# Autodesk Inventor assembly: CircuitCell
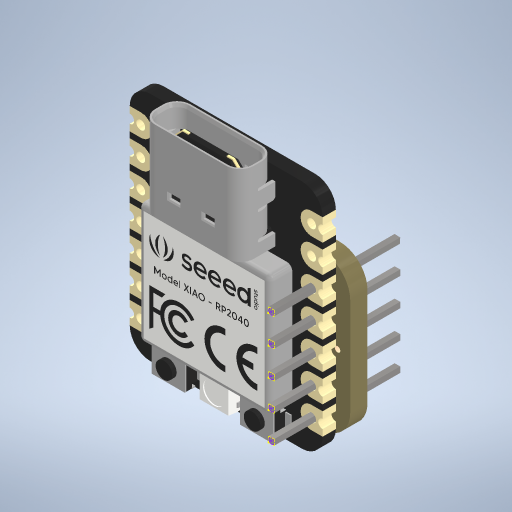
[picture p0: Inventor's stored thumbnail of the model, 512x512]
Saved by Autodesk Inventor 2023 (Build 270158000, 158)
## iProperties
Created: 2023-04-17
Part Number: CircuitCell
Document SubType Name: Assembly
Designer: maste
Author: maste
## Documents named in this file (4)
- C:\Users\maste\Documents\GitHub\Remote-Stethoscope\3D_models\ThonkLabs 1ne\SeparateDiaphragm\CircuitCell.iam
- C:\Users\maste\Documents\GitHub\Remote-Stethoscope\3D_models\Fall2022_revision\IC_pin.ipt
- C:\Users\maste\Documents\GitHub\Remote-Stethoscope\3D_models\adafruit_3492\PDM Mic.iam
- C:\Users\maste\Documents\GitHub\Remote-Stethoscope\3D_models\xiao_rp2040\Seeed Studio XIAO RP2040 v26.iam
## Components (7 placed, 3 different names)
1. IC_pin:1 — Mate:3, Flush:2, Flush:3, Flush:4, Flush:5, Flush:6, Mate:7
2. IC_pin:2 — Mate:2, Flush:3
3. IC_pin:3 — Mate:4, Flush:4
4. IC_pin:4 — Mate:5, Flush:5
5. IC_pin:5 — Mate:6, Flush:6
6. PDM Mic:1 [sub-assembly] — Mate:1, Mate:2, Mate:3, Mate:4, Mate:5, Mate:6, Flush:2, Angle:1
7. Seeed Studio XIAO RP2040 v26:1 [sub-assembly] — Mate:1, Mate:7, Angle:1
## Relationships (13: Mate 7, Flush 5, Angle 1)
- Mate:1: PDM Mic:1 ↔ Seeed Studio XIAO RP2040 v26:1
- Mate:2: IC_pin:2 ↔ PDM Mic:1
- Mate:3: IC_pin:1 ↔ PDM Mic:1
- Mate:4: IC_pin:3 ↔ PDM Mic:1
- Mate:5: IC_pin:4 ↔ PDM Mic:1
- Mate:6: IC_pin:5 ↔ PDM Mic:1
- Flush:2 (-5 mm): IC_pin:1 ↔ PDM Mic:1
- Flush:3: IC_pin:1 ↔ IC_pin:2
- Flush:4: IC_pin:1 ↔ IC_pin:3
- Flush:5: IC_pin:1 ↔ IC_pin:4
- Flush:6: IC_pin:1 ↔ IC_pin:5
- Mate:7: IC_pin:1 ↔ Seeed Studio XIAO RP2040 v26:1
- Angle:1 (0 deg): PDM Mic:1 ↔ Seeed Studio XIAO RP2040 v26:1
